# Autodesk Inventor assembly: completeCase
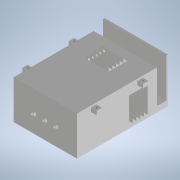
[picture p0: Inventor's stored thumbnail of the model, 180x180]
Saved by Autodesk Inventor 2022.6 (Build 266554010, 554A)
## iProperties
Created: 2025-03-20
Part Number: completeCase
Document SubType Name: Assembly
Designer: khinm
Author: khinm
## Documents named in this file (5)
- C:\Users\khinm\Downloads\CAD\completeCase.iam
- C:\Users\khinm\Downloads\CAD\caseDoor.ipt
- C:\Users\khinm\Downloads\CAD\rubberSeal.ipt
- C:\Users\khinm\Downloads\CAD\caseBody.ipt
- C:\Users\khinm\Downloads\CAD\basePlate.ipt
## Components (4 placed, 4 different names)
1. caseDoor:1 — Mate:1, Mate:2, Mate:3, Mate:4, Flush:1, Mate:6, Flush:2
2. rubberSeal:1 — Mate:1, Mate:2, Mate:3, Mate:4
3. caseBody:1 — Mate:5, Flush:1, Mate:6, Flush:2
4. basePlate:1 — Mate:5
## Relationships (8: Mate 6, Flush 2)
- Mate:1: caseDoor:1 ↔ rubberSeal:1
- Mate:2: caseDoor:1 ↔ rubberSeal:1
- Mate:3: caseDoor:1 ↔ rubberSeal:1
- Mate:4: caseDoor:1 ↔ rubberSeal:1
- Mate:5: caseBody:1 ↔ basePlate:1
- Flush:1: caseDoor:1 ↔ caseBody:1
- Mate:6: caseDoor:1 ↔ caseBody:1
- Flush:2: caseDoor:1 ↔ caseBody:1
